# Autodesk Inventor assembly: deformable mirror
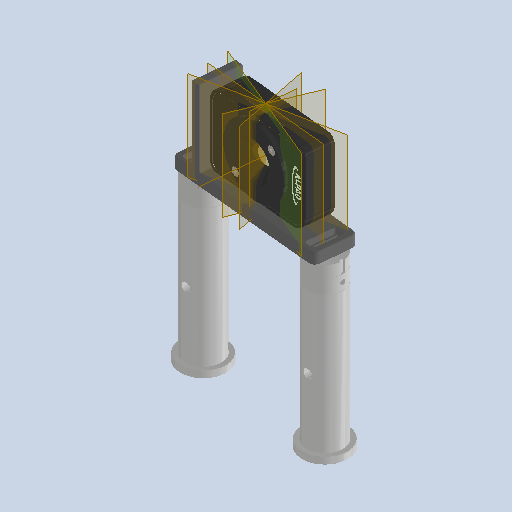
[picture p0: Inventor's stored thumbnail of the model, 512x512]
Saved by Autodesk Inventor 2026.1 (Build 301233000, 233)
## iProperties
Created: 2025-06-09
Part Number: deformable mirror
Document SubType Name: Assembly
Designer: Julian
Author: Julian
## Documents named in this file (6)
- C:\Users\user\Desktop\setup_inventor_2025\deformable mirror\deformable mirror.iam
- C:\Users\user\Desktop\setup_inventor_2025\deformable mirror\defmormable mirror mount.ipt
- C:\Users\user\Desktop\setup_inventor_2025\deformable mirror\DM06915005A.ipt
- C:\Users\user\Desktop\setup_inventor_2025\deformable mirror\RS10.ipt
- C:\Users\user\Desktop\setup_inventor_2025\deformable mirror\RS8.ipt
- C:\Users\user\Desktop\setup_inventor_2025\deformable mirror\RS4P.ipt
## Components (8 placed, 5 different names)
1. defmormable mirror mount:1 — Passend:1, Passend:2, Passend:3, Passend:12, Passend:13, Passend:14, Passend:15, Passend:16, Passend:17
2. DM06915005A:1 — Passend:1, Passend:2, Passend:3
3. RS10:1 — Passend:4, Passend:10, Passend:11
4. RS10:2 — Passend:6, Passend:8, Passend:9
5. RS8:1 — Passend:7, Passend:9, Passend:13, Passend:14, Passend:16
6. RS8:2 — Passend:5, Passend:11, Passend:12, Passend:15, Passend:17
7. RS4P:1 — Passend:4, Passend:5, Passend:10
8. RS4P:2 — Passend:6, Passend:7, Passend:8
## Relationships (17: Mate 17)
- Passend:1 [Mate]: defmormable mirror mount:1 ↔ DM06915005A:1
- Passend:2 [Mate]: defmormable mirror mount:1 ↔ DM06915005A:1
- Passend:3 [Mate]: defmormable mirror mount:1 ↔ DM06915005A:1
- Passend:4 [Mate]: RS10:1 ↔ RS4P:1
- Passend:5 [Mate]: RS8:2 ↔ RS4P:1
- Passend:6 [Mate]: RS10:2 ↔ RS4P:2
- Passend:7 [Mate]: RS8:1 ↔ RS4P:2
- Passend:8 [Mate]: RS10:2 ↔ RS4P:2
- Passend:9 [Mate]: RS10:2 ↔ RS8:1
- Passend:10 [Mate]: RS10:1 ↔ RS4P:1
- Passend:11 [Mate]: RS10:1 ↔ RS8:2
- Passend:12 [Mate]: defmormable mirror mount:1 ↔ RS8:2
- Passend:13 [Mate]: defmormable mirror mount:1 ↔ RS8:1
- Passend:14 [Mate] (2 mm): defmormable mirror mount:1 ↔ RS8:1
- Passend:15 [Mate] (10 mm): defmormable mirror mount:1 ↔ RS8:2
- Passend:16 [Mate] (10 mm): defmormable mirror mount:1 ↔ RS8:1
- Passend:17 [Mate] (2 mm): defmormable mirror mount:1 ↔ RS8:2
